# Autodesk Inventor assembly: Assembly_Cube_Lightsheet_Sample_v3
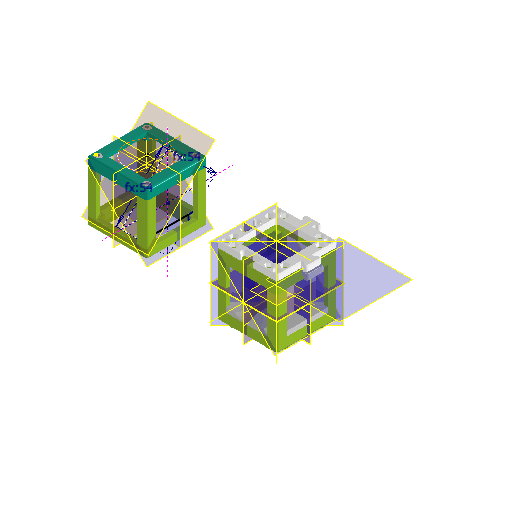
[picture p0: Inventor's stored thumbnail of the model, 512x512]
Saved by Autodesk Inventor 2025.1 (Build 291241020, 241B)
## iProperties
Created: 2023-03-07
Part Number: Assembly_Cube_Lightsheet_Sample_v3
Document SubType Name: Assembly
Designer: diederichbenedict
Author: diederichbenedict
## Documents named in this file (4)
- C:\Users\diederichbenedict\Dropbox\Dokumente\Promotion\PROJECTS\openUC2-CAD\INVENTOR\Assembly_Cube_Lightsheet_Sample_v3.iam
- C:\Users\diederichbenedict\Dropbox\Dokumente\Promotion\PROJECTS\openUC2-CAD\INVENTOR\20_Cube_Insert_Lightsheet_FEPTube_Pipette_v3.ipt
- C:\Users\diederichbenedict\Dropbox\Dokumente\Promotion\PROJECTS\openUC2-CAD\INVENTOR\Assembly_Cube_empty_IM_v3.iam
- C:\Users\diederichbenedict\Dropbox\Dokumente\Promotion\PROJECTS\openUC2-CAD\INVENTOR\Assembly_Cube_empty_1x1_v3.iam
## Components (3 placed, 3 different names)
1. Assembly_Cube_empty_IM_v3:1 [sub-assembly] — Mate:1, Mate:2, Mate:3
2. 20_Cube_Insert_Lightsheet_FEPTube_Pipette_v3:1 — Mate:1, Mate:2, Mate:3
3. Assembly_Cube_empty_1x1_v3:1 [sub-assembly]
## Relationships (3: Mate 3)
- Mate:1: Assembly_Cube_empty_IM_v3:1 ↔ 20_Cube_Insert_Lightsheet_FEPTube_Pipette_v3:1
- Mate:2: Assembly_Cube_empty_IM_v3:1 ↔ 20_Cube_Insert_Lightsheet_FEPTube_Pipette_v3:1
- Mate:3: Assembly_Cube_empty_IM_v3:1 ↔ 20_Cube_Insert_Lightsheet_FEPTube_Pipette_v3:1
